# Autodesk Inventor assembly: assem_thumb_v1
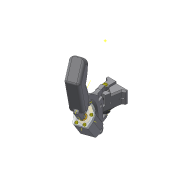
[picture p0: Inventor's stored thumbnail of the model, 180x180]
Saved by Autodesk Inventor 2014 (Build 180170000, 170)
## iProperties
Created: 2015-07-28
Part Number: assem_thumb_v1
Document SubType Name: Assembly
Designer: Martin
Author: Martin
## Documents named in this file (14)
- C:\Users\Martin\Dropbox\biohand-mec\biohand_v1\fingers\thumb\assem_thumb_v1.iam
- C:\Users\Martin\Dropbox\biohand-mec\biohand_v1\palm\servo_clamp_v2.ipt
- C:\Users\Martin\Dropbox\biohand-mec\biohand_v1\misc\bearing_10_4_3.ipt
- C:\Users\Martin\Dropbox\biohand-mec\biohand_v1\misc\micro_servo.ipt
- C:\Users\Martin\Dropbox\biohand-mec\biohand_v1\fingers\thumb\thumb_base_v2.ipt
- C:\Users\Martin\Dropbox\biohand-mec\biohand_v1\misc\m2_4_screw.ipt
- C:\Users\Martin\Dropbox\biohand-mec\biohand_v1\misc\m2_8_screw.ipt
- C:\Users\Martin\Dropbox\biohand-mec\biohand_v1\misc\m3_10_screw.ipt
- C:\Users\Martin\Dropbox\biohand-mec\biohand_v1\fingers\thumb\assem_finger_thumb_linact_v3.iam
- C:\Users\Martin\Dropbox\biohand-mec\biohand_v1\fingers\thumb\linact_thumb_rod.ipt
- C:\Users\Martin\Dropbox\biohand-mec\biohand_v1\misc\m3_nut.ipt
- C:\Users\Martin\Dropbox\biohand-mec\biohand_v1\fingers\thumb\thumb_phalanx_v2_a.ipt
- C:\Users\Martin\Dropbox\biohand-mec\biohand_v1\misc\servo_square_pot.ipt
- C:\Users\Martin\Dropbox\biohand-mec\biohand_v1\misc\servo_hub_simple.ipt
## Components (15 placed, 13 different names)
1. servo_clamp_v2:1 — Flush:1, Mate:1, Flush:2, Insert:1, Mate:2, Mate:3, Angle:1, Mate:4, Mate:5
2. bearing_10_4_3:1 — Insert:1
3. micro_servo:1 — Mate:2, Mate:3, Angle:1, Insert:2, Insert:3, Insert:11
4. thumb_base_v2:1 — Mate:4, Insert:4, Mate:5, Insert:5, Insert:9, Angle:3
5. m2_4_screw:1 — Insert:2
6. m2_8_screw:1 — Insert:3
7. m3_10_screw:1 — Insert:4
8. assem_finger_thumb_linact_v3:1 [sub-assembly] — Insert:5, Mate:7, Flush:3
9. linact_thumb_rod:1 — Insert:6, Mate:6, Insert:7, Insert:8, Mate:7, Flush:3, Mate:8
10. m3_nut:1 — Insert:6, Mate:6
11. m2_4_screw:2 — Insert:8
12. m2_8_screw:2 — Insert:7
13. thumb_phalanx_v2_a:1 — Insert:9, Mate:8, Insert:10, Angle:2
14. servo_square_pot:1 — Insert:10, Angle:2
15. servo_hub_simple:1 — Insert:11, Angle:3
## Relationships (25: Insert 11, Mate 8, Flush 3, Angle 3)
- Flush:1: servo_clamp_v2:1
- Mate:1: servo_clamp_v2:1
- Flush:2: servo_clamp_v2:1
- Insert:1: servo_clamp_v2:1 ↔ bearing_10_4_3:1
- Mate:2: servo_clamp_v2:1 ↔ micro_servo:1
- Mate:3: servo_clamp_v2:1 ↔ micro_servo:1
- Angle:1 (0 deg): servo_clamp_v2:1 ↔ micro_servo:1
- Mate:4: servo_clamp_v2:1 ↔ thumb_base_v2:1
- Insert:2: micro_servo:1 ↔ m2_4_screw:1
- Insert:3: micro_servo:1 ↔ m2_8_screw:1
- Insert:4: thumb_base_v2:1 ↔ m3_10_screw:1
- Mate:5 (2 mm): servo_clamp_v2:1 ↔ thumb_base_v2:1
- Insert:5 (0.5 mm): thumb_base_v2:1 ↔ assem_finger_thumb_linact_v3:1
- Insert:6: linact_thumb_rod:1 ↔ m3_nut:1
- Mate:6: linact_thumb_rod:1 ↔ m3_nut:1
- Insert:7: linact_thumb_rod:1 ↔ m2_8_screw:2
- Insert:8: linact_thumb_rod:1 ↔ m2_4_screw:2
- Mate:7: assem_finger_thumb_linact_v3:1 ↔ linact_thumb_rod:1
- Flush:3: assem_finger_thumb_linact_v3:1 ↔ linact_thumb_rod:1
- Insert:9 (0.5 mm): thumb_base_v2:1 ↔ thumb_phalanx_v2_a:1
- Mate:8: linact_thumb_rod:1 ↔ thumb_phalanx_v2_a:1
- Insert:10: thumb_phalanx_v2_a:1 ↔ servo_square_pot:1
- Angle:2 (180 deg): thumb_phalanx_v2_a:1 ↔ servo_square_pot:1
- Insert:11 (1.55 mm): micro_servo:1 ↔ servo_hub_simple:1
- Angle:3 (0 deg): thumb_base_v2:1 ↔ servo_hub_simple:1
